# Autodesk Inventor assembly: Cart Assembly
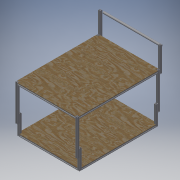
[picture p0: Inventor's stored thumbnail of the model, 180x180]
Saved by Autodesk Inventor 2016 SP2 (Build 200236200, 236)
## iProperties
Created: 2018-02-07
Part Number: Cart Assembly
Document SubType Name: Assembly
Designer: CAD
Author: CAD
## Documents named in this file (10)
- C:\Users\CAD\Documents\GitHub\FIRST-ROBOTICS-2018-5436-CAD\Cart\Cart Assembly.iam
- C:\Users\CAD\Documents\GitHub\FIRST-ROBOTICS-2018-5436-CAD\Cart\Horizontal width piece.ipt
- C:\Users\CAD\Documents\GitHub\FIRST-ROBOTICS-2018-5436-CAD\Cart\Horizontal pice.ipt
- C:\Users\CAD\Documents\GitHub\FIRST-ROBOTICS-2018-5436-CAD\Cart\Vertical piece Handle side.ipt
- C:\Users\CAD\Documents\GitHub\FIRST-ROBOTICS-2018-5436-CAD\Cart\cart plywood.ipt
- C:\Users\CAD\Documents\GitHub\FIRST-ROBOTICS-2018-5436-CAD\Cart\Outside side vertical.ipt
- C:\Users\CAD\Documents\GitHub\FIRST-ROBOTICS-2018-5436-CAD\Cart\cart plywood top side.ipt
- C:\Users\CAD\Documents\GitHub\FIRST-ROBOTICS-2018-5436-CAD\Cart\Horizontal piceTOP.ipt
- C:\Users\CAD\Documents\GitHub\FIRST-ROBOTICS-2018-5436-CAD\Cart\Handle Holding PIECE.ipt
- C:\Users\CAD\Documents\GitHub\FIRST-ROBOTICS-2018-5436-CAD\Cart\Handle.ipt
## Components (25 placed, 9 different names)
1. Horizontal width piece:2 — Flush:4, Flush:8, Flush:29, Mate:22, Mate:23, Flush:30, Flush:32, Mate:54
2. Horizontal pice:1 — Flush:4, Mate:11, Mate:20, Flush:35, Mate:28, Flush:39, Mate:51, Mate:53
3. Horizontal pice:2 — Flush:8, Mate:5, Flush:9, Flush:10, Mate:24, Flush:31
4. Vertical piece Handle side:1 — Mate:5, Flush:9, Flush:10, Mate:30, Mate:44, Flush:45, Mate:49
5. cart plywood:1 — Mate:11, Mate:26, Flush:36, Mate:50, Mate:52
6. Vertical piece Handle side:3 — Mate:23, Mate:24, Flush:30, Flush:31, Flush:33, Mate:26, Mate:43, Flush:43, Mate:48
7. Vertical piece Handle side:4 — Mate:20, Flush:29, Mate:22, Flush:32, Flush:33, Flush:35, Flush:36, Mate:42, Flush:42
8. Vertical piece Handle side:5 — Mate:28, Mate:29, Flush:38, Flush:39, Flush:40, Flush:47, Mate:45
9. Horizontal width piece:7 — Mate:29, Flush:38, Flush:40, Mate:30
10. Outside side vertical:1 — Mate:43, Flush:43, Flush:44, Flush:50, Mate:60, Flush:53
11. Outside side vertical:2 — Mate:42, Flush:42, Flush:44, Flush:46, Flush:48, Flush:51, Mate:56, Mate:63, Flush:54
12. Outside side vertical:3 — Mate:44, Flush:45, Flush:46, Mate:46, Flush:49, Mate:49, Flush:52, Flush:56, Mate:71
13. Outside side vertical:4 — Flush:47, Mate:45, Flush:48, Mate:58, Mate:70, Flush:55, Mate:72
14. cart plywood top side:1 — Mate:46, Flush:49, Flush:50, Mate:48, Mate:57, Mate:59, Mate:61, Mate:62, Mate:65, Mate:66
15. Horizontal width piece:8 — Flush:51, Mate:56, Mate:57
16. Horizontal width piece:9 — Mate:58, Flush:52, Mate:59, Mate:68
17. Horizontal width piece:10 — Mate:64, Mate:65, Mate:69
18. Horizontal width piece:11 — Mate:66, Mate:67, Mate:68, Mate:69
19. Horizontal width piece:12 — Mate:52, Mate:53, Mate:54, Mate:55
20. Horizontal width piece:13 — Mate:50, Mate:51, Mate:55
21. Horizontal piceTOP:1 — Mate:62, Mate:63, Flush:54
22. Horizontal piceTOP:2 — Mate:60, Mate:61, Flush:53, Mate:64, Mate:67
23. Handle Holding PIECE:1 — Mate:70, Flush:55, Flush:57, Mate:72, Mate:73
24. Handle Holding PIECE:2 — Flush:56, Mate:71, Flush:57
25. Handle:1 — Mate:73
## Relationships (71: Mate 41, Flush 30)
- Flush:4: Horizontal width piece:2 ↔ Horizontal pice:1
- Flush:8: Horizontal width piece:2 ↔ Horizontal pice:2
- Mate:5: Horizontal pice:2 ↔ Vertical piece Handle side:1
- Flush:9: Horizontal pice:2 ↔ Vertical piece Handle side:1
- Flush:10: Horizontal pice:2 ↔ Vertical piece Handle side:1
- Mate:11: Horizontal pice:1 ↔ cart plywood:1
- Mate:20: Horizontal pice:1 ↔ Vertical piece Handle side:4
- Flush:29: Horizontal width piece:2 ↔ Vertical piece Handle side:4
- Mate:22: Horizontal width piece:2 ↔ Vertical piece Handle side:4
- Mate:23: Horizontal width piece:2 ↔ Vertical piece Handle side:3
- Mate:24: Horizontal pice:2 ↔ Vertical piece Handle side:3
- Flush:30: Horizontal width piece:2 ↔ Vertical piece Handle side:3
- Flush:31: Horizontal pice:2 ↔ Vertical piece Handle side:3
- Flush:32: Horizontal width piece:2 ↔ Vertical piece Handle side:4
- Flush:33: Vertical piece Handle side:3 ↔ Vertical piece Handle side:4
- Mate:26: cart plywood:1 ↔ Vertical piece Handle side:3
- Flush:35: Horizontal pice:1 ↔ Vertical piece Handle side:4
- Flush:36: cart plywood:1 ↔ Vertical piece Handle side:4
- Mate:28: Horizontal pice:1 ↔ Vertical piece Handle side:5
- Mate:29: Vertical piece Handle side:5 ↔ Horizontal width piece:7
- Flush:38: Vertical piece Handle side:5 ↔ Horizontal width piece:7
- Flush:39: Horizontal pice:1 ↔ Vertical piece Handle side:5
- Flush:40: Vertical piece Handle side:5 ↔ Horizontal width piece:7
- Mate:30: Vertical piece Handle side:1 ↔ Horizontal width piece:7
- Mate:42: Vertical piece Handle side:4 ↔ Outside side vertical:2
- Flush:42: Vertical piece Handle side:4 ↔ Outside side vertical:2
- Mate:43: Vertical piece Handle side:3 ↔ Outside side vertical:1
- Flush:43: Vertical piece Handle side:3 ↔ Outside side vertical:1
- Flush:44: Outside side vertical:1 ↔ Outside side vertical:2
- Mate:44: Vertical piece Handle side:1 ↔ Outside side vertical:3
- Flush:45: Vertical piece Handle side:1 ↔ Outside side vertical:3
- Flush:46: Outside side vertical:2 ↔ Outside side vertical:3
- Flush:47: Vertical piece Handle side:5 ↔ Outside side vertical:4
- Mate:45: Vertical piece Handle side:5 ↔ Outside side vertical:4
- Flush:48: Outside side vertical:2 ↔ Outside side vertical:4
- Mate:46: Outside side vertical:3 ↔ cart plywood top side:1
- Flush:49: Outside side vertical:3 ↔ cart plywood top side:1
- Flush:50: Outside side vertical:1 ↔ cart plywood top side:1
- Mate:48: Vertical piece Handle side:3 ↔ cart plywood top side:1
- Mate:49: Vertical piece Handle side:1 ↔ Outside side vertical:3
- Mate:50: cart plywood:1 ↔ Horizontal width piece:13
- Mate:51: Horizontal pice:1 ↔ Horizontal width piece:13
- Mate:52: cart plywood:1 ↔ Horizontal width piece:12
- Mate:53: Horizontal pice:1 ↔ Horizontal width piece:12
- Mate:54 (287.8667 mm): Horizontal width piece:2 ↔ Horizontal width piece:12
- Mate:55 (287.8667 mm): Horizontal width piece:12 ↔ Horizontal width piece:13
- Flush:51: Outside side vertical:2 ↔ Horizontal width piece:8
- Mate:56: Outside side vertical:2 ↔ Horizontal width piece:8
- Mate:57: cart plywood top side:1 ↔ Horizontal width piece:8
- Mate:58: Outside side vertical:4 ↔ Horizontal width piece:9
- Flush:52: Outside side vertical:3 ↔ Horizontal width piece:9
- Mate:59: cart plywood top side:1 ↔ Horizontal width piece:9
- Mate:60: Outside side vertical:1 ↔ Horizontal piceTOP:2
- Mate:61: cart plywood top side:1 ↔ Horizontal piceTOP:2
- Flush:53: Outside side vertical:1 ↔ Horizontal piceTOP:2
- Mate:62: cart plywood top side:1 ↔ Horizontal piceTOP:1
- Mate:63: Outside side vertical:2 ↔ Horizontal piceTOP:1
- Flush:54: Outside side vertical:2 ↔ Horizontal piceTOP:1
- Mate:64: Horizontal width piece:10 ↔ Horizontal piceTOP:2
- Mate:65: cart plywood top side:1 ↔ Horizontal width piece:10
- Mate:66: cart plywood top side:1 ↔ Horizontal width piece:11
- Mate:67: Horizontal width piece:11 ↔ Horizontal piceTOP:2
- Mate:68 (287.8667 mm): Horizontal width piece:9 ↔ Horizontal width piece:11
- Mate:69 (287.8667 mm): Horizontal width piece:10 ↔ Horizontal width piece:11
- Mate:70: Outside side vertical:4 ↔ Handle Holding PIECE:1
- Flush:55: Outside side vertical:4 ↔ Handle Holding PIECE:1
- Flush:56: Outside side vertical:3 ↔ Handle Holding PIECE:2
- Mate:71: Outside side vertical:3 ↔ Handle Holding PIECE:2
- Flush:57: Handle Holding PIECE:1 ↔ Handle Holding PIECE:2
- Mate:72 (-50.8 mm): Outside side vertical:4 ↔ Handle Holding PIECE:1
- Mate:73: Handle Holding PIECE:1 ↔ Handle:1
